# Autodesk Inventor assembly: HbSocketU02
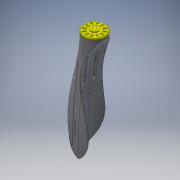
[picture p0: Inventor's stored thumbnail of the model, 180x180]
Saved by Autodesk Inventor 2016 (Build 200138000, 138)
## iProperties
Created: 2015-02-09
Part Number: HbSocketU02
Document SubType Name: Assembly
Designer: Yamaura
Author: Yamaura
## Documents named in this file (19)
- C:\Users\Yamaura\Documents\GitHub\HACKberry\HACKberry-hardware\3D\Inventor\Parts\HbSocketU02.iam
- C:\Users\Yamaura\Documents\GitHub\HACKberry\HACKberry-hardware\3D\Inventor\Parts\HbBatteryDoor03.ipt
- C:\Users\Yamaura\Documents\GitHub\HACKberry\HACKberry-hardware\3D\Inventor\Parts\HbBatteryDoorKnob03.ipt
- C:\Users\Yamaura\Documents\GitHub\HACKberry\HACKberry-hardware\3D\Inventor\Parts\HbBatteryHingeA03.ipt
- C:\Users\Yamaura\Documents\GitHub\HACKberry\HACKberry-hardware\3D\Inventor\Parts\HbBatteryHingeB03.ipt
- C:\Users\Yamaura\Documents\GitHub\HACKberry\HACKberry-hardware\3D\Inventor\Parts\HbBatteryHingeC03.ipt
- C:\Users\Yamaura\Documents\GitHub\HACKberry\HACKberry-hardware\3D\Inventor\Parts\HbBatteryCase01.ipt
- C:\Users\Yamaura\Documents\GitHub\HACKberry\HACKberry-hardware\3D\Inventor\Parts\HbBatteryLockKnob01.ipt
- C:\Users\Yamaura\Documents\GitHub\HACKberry\HACKberry-hardware\3D\Inventor\Parts\DMW-BLF19.ipt
- C:\Users\Yamaura\Documents\GitHub\HACKberry\HACKberry-hardware\3D\Inventor\Parts\HbBatteryDoorLever03.ipt
- C:\Users\Yamaura\Documents\GitHub\HACKberry\HACKberry-hardware\3D\Inventor\Parts\HbMainFrameA01.ipt
- C:\Users\Yamaura\Documents\GitHub\HACKberry\HACKberry-hardware\3D\Inventor\Parts\HbMainFrameB01.ipt
- C:\Users\Yamaura\Documents\GitHub\HACKberry\HACKberry-hardware\3D\Inventor\Parts\TS 0.4-3.2-14.ipt
- C:\Users\Yamaura\Documents\GitHub\HACKberry\HACKberry-hardware\3D\Inventor\Parts\flatScrewM2L6PHI3.3T1.3.ipt
- C:\Users\Yamaura\Documents\GitHub\HACKberry\HACKberry-hardware\3D\Inventor\Parts\101050-003.ipt
- C:\Users\Yamaura\Documents\GitHub\HACKberry\HACKberry-hardware\3D\Inventor\Parts\HbBatteryPcb02.ipt
- C:\Users\Yamaura\Documents\GitHub\HACKberry\HACKberry-hardware\3D\Inventor\Parts\CP 0.5-6-8.ipt
- C:\Users\Yamaura\Documents\GitHub\HACKberry\HACKberry-hardware\3D\Inventor\Parts\HbPowerWire+7.2V.ipt
- C:\Users\Yamaura\Documents\GitHub\HACKberry\HACKberry-hardware\3D\Inventor\Parts\HbWristLockPlate01.ipt
## Components (25 placed, 18 different names)
1. HbBatteryCase01:1 — フラッシュ:15, フラッシュ:17, メイト:78, メイト:80, メイト:81, メイト:85, メイト:91, フラッシュ:18, メイト:92, フラッシュ:19, フラッシュ:20, フラッシュ:21, メイト:93, メイト:94, メイト:95, メイト:96, フラッシュ:23
2. HbBatteryLockKnob01:1 — メイト:95, メイト:97
3. DMW-BLF19:1 — メイト:78, メイト:79, メイト:80
4. flatScrewM2L6PHI3.3T1.3:1 — フラッシュ:18, メイト:92
5. flatScrewM2L6PHI3.3T1.3:2 — フラッシュ:21, メイト:93
6. flatScrewM2L6PHI3.3T1.3:3 — フラッシュ:20, メイト:94
7. flatScrewM2L6PHI3.3T1.3:4 — フラッシュ:19, メイト:96
8. TS 0.4-3.2-14:1 — メイト:73, 正接:1, 正接:2, 正接:3
9. HbBatteryHingeC03:1 — メイト:49, メイト:50, メイト:51
10. HbBatteryHingeB03:1 — メイト:45, メイト:47, メイト:102, メイト:103
11. HbBatteryHingeA03:1 — メイト:44, メイト:46, メイト:101
12. HbBatteryDoor03:1 — メイト:44, メイト:45, メイト:46, メイト:47, メイト:49, メイト:50, メイト:51, メイト:102
13. HbMainFrameA01:1 — フラッシュ:6, フラッシュ:7, フラッシュ:8, メイト:73, 正接:1, 正接:2, メイト:75, メイト:76, メイト:104, メイト:105, メイト:106
14. HbBatteryDoorKnob03:3 — メイト:58, メイト:59, メイト:60, 正接:3
15. HbMainFrameB01:1 — フラッシュ:14, メイト:75, メイト:76, メイト:90, メイト:97, メイト:98, メイト:99, メイト:100, フラッシュ:24, メイト:101, メイト:103
16. 101050-003:1 — メイト:88, メイト:89
17. 101050-003:2 — メイト:81, メイト:86, メイト:87
18. HbBatteryPcb02:1 — メイト:85, メイト:86, メイト:87, メイト:88, メイト:89, メイト:90, メイト:91, メイト:100, フラッシュ:22, フラッシュ:25, フラッシュ:26, フラッシュ:27
19. CP 0.5-6-8:1 — メイト:98, メイト:99
20. HbPowerWire+7.2V:1 — フラッシュ:22, フラッシュ:23, フラッシュ:24, フラッシュ:25, フラッシュ:26, フラッシュ:27
21. HbWristLockPlate01:1 — メイト:104, メイト:105, メイト:106
22. HbBatteryDoorKnob03:1 — メイト:37, メイト:38, メイト:39
23. HbBatteryDoorKnob03:2
24. HbBatteryDoorLever03:1 — メイト:37, メイト:38, メイト:39, メイト:58, メイト:59, メイト:60
25. HbBatteryDoorLever03:2
## Component patterns: (2 elements, first: HbBatteryDoorKnob03:1), (2 elements, first: HbBatteryDoorLever03:1)
## Relationships (62: Mate 42, Flush 17, Tangent 3)
- メイト:37 [Mate]: HbBatteryDoorKnob03:1 ↔ HbBatteryDoorLever03:1
- メイト:38 [Mate]: HbBatteryDoorKnob03:1 ↔ HbBatteryDoorLever03:1
- メイト:39 [Mate]: HbBatteryDoorKnob03:1 ↔ HbBatteryDoorLever03:1
- メイト:44 [Mate]: HbBatteryHingeA03:1 ↔ HbBatteryDoor03:1
- メイト:45 [Mate]: HbBatteryHingeB03:1 ↔ HbBatteryDoor03:1
- メイト:46 [Mate]: HbBatteryHingeA03:1 ↔ HbBatteryDoor03:1
- メイト:47 [Mate]: HbBatteryHingeB03:1 ↔ HbBatteryDoor03:1
- メイト:49 [Mate]: HbBatteryHingeC03:1 ↔ HbBatteryDoor03:1
- メイト:50 [Mate]: HbBatteryHingeC03:1 ↔ HbBatteryDoor03:1
- メイト:51 [Mate]: HbBatteryHingeC03:1 ↔ HbBatteryDoor03:1
- フラッシュ:6 [Flush] (-0.2 mm): HbMainFrameA01:1
- フラッシュ:7 [Flush]: HbMainFrameA01:1
- フラッシュ:8 [Flush]: HbMainFrameA01:1
- メイト:58 [Mate]: HbBatteryDoorKnob03:3 ↔ HbBatteryDoorLever03:1
- メイト:59 [Mate]: HbBatteryDoorKnob03:3 ↔ HbBatteryDoorLever03:1
- メイト:60 [Mate]: HbBatteryDoorKnob03:3 ↔ HbBatteryDoorLever03:1
- メイト:73 [Mate] (-2.4 mm): TS 0.4-3.2-14:1 ↔ HbMainFrameA01:1
- 正接:1 [Tangent]: TS 0.4-3.2-14:1 ↔ HbMainFrameA01:1
- 正接:2 [Tangent]: TS 0.4-3.2-14:1 ↔ HbMainFrameA01:1
- 正接:3 [Tangent]: TS 0.4-3.2-14:1 ↔ HbBatteryDoorKnob03:3
- フラッシュ:14 [Flush]: HbMainFrameB01:1
- メイト:75 [Mate]: HbMainFrameA01:1 ↔ HbMainFrameB01:1
- メイト:76 [Mate] (0.2 mm): HbMainFrameA01:1 ↔ HbMainFrameB01:1
- フラッシュ:15 [Flush]: HbBatteryCase01:1
- フラッシュ:16 [Flush] (-224 mm)
- フラッシュ:17 [Flush]: HbBatteryCase01:1
- メイト:78 [Mate]: HbBatteryCase01:1 ↔ DMW-BLF19:1
- メイト:79 [Mate]: DMW-BLF19:1
- メイト:80 [Mate]: HbBatteryCase01:1 ↔ DMW-BLF19:1
- メイト:81 [Mate]: HbBatteryCase01:1 ↔ 101050-003:2
- メイト:85 [Mate]: HbBatteryCase01:1 ↔ HbBatteryPcb02:1
- メイト:86 [Mate]: 101050-003:2 ↔ HbBatteryPcb02:1
- メイト:87 [Mate]: 101050-003:2 ↔ HbBatteryPcb02:1
- メイト:88 [Mate]: 101050-003:1 ↔ HbBatteryPcb02:1
- メイト:89 [Mate]: 101050-003:1 ↔ HbBatteryPcb02:1
- メイト:90 [Mate]: HbMainFrameB01:1 ↔ HbBatteryPcb02:1
- メイト:91 [Mate]: HbBatteryCase01:1 ↔ HbBatteryPcb02:1
- フラッシュ:18 [Flush]: HbBatteryCase01:1 ↔ flatScrewM2L6PHI3.3T1.3:1
- メイト:92 [Mate]: HbBatteryCase01:1 ↔ flatScrewM2L6PHI3.3T1.3:1
- フラッシュ:19 [Flush]: HbBatteryCase01:1 ↔ flatScrewM2L6PHI3.3T1.3:4
- フラッシュ:20 [Flush]: HbBatteryCase01:1 ↔ flatScrewM2L6PHI3.3T1.3:3
- フラッシュ:21 [Flush]: HbBatteryCase01:1 ↔ flatScrewM2L6PHI3.3T1.3:2
- メイト:93 [Mate]: HbBatteryCase01:1 ↔ flatScrewM2L6PHI3.3T1.3:2
- メイト:94 [Mate]: HbBatteryCase01:1 ↔ flatScrewM2L6PHI3.3T1.3:3
- メイト:95 [Mate]: HbBatteryCase01:1 ↔ HbBatteryLockKnob01:1
- メイト:96 [Mate]: HbBatteryCase01:1 ↔ flatScrewM2L6PHI3.3T1.3:4
- メイト:97 [Mate]: HbBatteryLockKnob01:1 ↔ HbMainFrameB01:1
- メイト:98 [Mate]: HbMainFrameB01:1 ↔ CP 0.5-6-8:1
- メイト:99 [Mate]: HbMainFrameB01:1 ↔ CP 0.5-6-8:1
- メイト:100 [Mate]: HbMainFrameB01:1 ↔ HbBatteryPcb02:1
- フラッシュ:22 [Flush]: HbBatteryPcb02:1 ↔ HbPowerWire+7.2V:1
- フラッシュ:23 [Flush]: HbBatteryCase01:1 ↔ HbPowerWire+7.2V:1
- フラッシュ:24 [Flush]: HbMainFrameB01:1 ↔ HbPowerWire+7.2V:1
- フラッシュ:25 [Flush]: HbBatteryPcb02:1 ↔ HbPowerWire+7.2V:1
- フラッシュ:26 [Flush]: HbBatteryPcb02:1 ↔ HbPowerWire+7.2V:1
- フラッシュ:27 [Flush]: HbBatteryPcb02:1 ↔ HbPowerWire+7.2V:1
- メイト:101 [Mate]: HbBatteryHingeA03:1 ↔ HbMainFrameB01:1
- メイト:102 [Mate]: HbBatteryHingeB03:1 ↔ HbBatteryDoor03:1
- メイト:103 [Mate]: HbBatteryHingeB03:1 ↔ HbMainFrameB01:1
- メイト:104 [Mate]: HbMainFrameA01:1 ↔ HbWristLockPlate01:1
- メイト:105 [Mate]: HbMainFrameA01:1 ↔ HbWristLockPlate01:1
- メイト:106 [Mate]: HbMainFrameA01:1 ↔ HbWristLockPlate01:1
